# Autodesk Inventor assembly: Egg Capsule ver 2
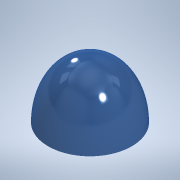
[picture p0: Inventor's stored thumbnail of the model, 180x180]
Saved by Autodesk Inventor 2022 (Build 260153000, 153)
## iProperties
Created: 2022-02-15
Part Number: Egg Capsule ver 2
Document SubType Name: Assembly
Designer: Nathan Griffith
Author: Nathan Griffith
## Documents named in this file (4)
- C:\Users\Nathan Griffith\Documents\Inventor\Physics Egg Drop\Egg Capsule ver 2.iam
- C:\Users\Nathan Griffith\Documents\Inventor\Physics Egg Drop\Egg Capsule Top.ipt
- C:\Users\Nathan Griffith\Documents\Inventor\Physics Egg Drop\Egg Rubber Inside Top.ipt
- C:\Users\Nathan Griffith\Documents\Inventor\Physics Egg Drop\Rubber Cover Top.ipt
## Components (3 placed, 3 different names)
1. Egg Capsule Top:1 — Insert:1, Insert:2, Insert:3
2. Egg Rubber Inside Top:1 — Insert:1
3. Rubber Cover Top:1 — Insert:2, Insert:3
## Relationships (3: Insert 3)
- Insert:1: Egg Capsule Top:1 ↔ Egg Rubber Inside Top:1
- Insert:2: Egg Capsule Top:1 ↔ Rubber Cover Top:1
- Insert:3: Egg Capsule Top:1 ↔ Rubber Cover Top:1
